# Autodesk Inventor assembly: POM_T5_03
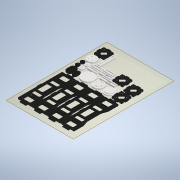
[picture p0: Inventor's stored thumbnail of the model, 180x180]
Saved by Autodesk Inventor 2020 (Build 240168000, 168)
## iProperties
Created: 2021-08-27
Part Number: POM_T5_03
Document SubType Name: Assembly
Designer: Masato
Author: Masato
## Documents named in this file (20)
- C:\Users\naoki\Documents\Inventor\CitBrains\git_clone\SUSTAINA_ver1_0\治具\SUSTAINA-OP\Cam\POM_T5_03.iam
- C:\Users\naoki\Documents\Inventor\CitBrains\git_clone\SUSTAINA_ver1_0\GFRP\SUSTAINA-OP\Cam\DisposableBoard.ipt
- C:\Users\naoki\Documents\Inventor\CitBrains\git_clone\SUSTAINA_ver1_0\GFRP\SUSTAINA-OP\UpperBody\Trunk\Trunk_chest_frame.ipt
- C:\Users\naoki\Documents\Inventor\CitBrains\git_clone\SUSTAINA_ver1_0\治具\SUSTAINA-OP\SandBlastingJig\Foot_front_frame_SandBlastingJig_back.ipt
- C:\Users\naoki\Documents\Inventor\CitBrains\git_clone\SUSTAINA_ver1_0\治具\SUSTAINA-OP\SandBlastingJig\Foot_front_frame_SandBlastingJig_front.ipt
- C:\Users\naoki\Documents\Inventor\CitBrains\git_clone\SUSTAINA_ver1_0\治具\SUSTAINA-OP\SandBlastingJig\Leg_joint_slider_frame_SandBlastingJig_axis_back.ipt
- C:\Users\naoki\Documents\Inventor\CitBrains\git_clone\SUSTAINA_ver1_0\治具\SUSTAINA-OP\SandBlastingJig\Leg_joint_slider_frame_SandBlastingJig_axis_front.ipt
- C:\Users\naoki\Documents\Inventor\CitBrains\git_clone\SUSTAINA_ver1_0\治具\SUSTAINA-OP\SandBlastingJig\Leg_joint_slider_frame_SandBlastingJig_slider_back.ipt
- C:\Users\naoki\Documents\Inventor\CitBrains\git_clone\SUSTAINA_ver1_0\治具\SUSTAINA-OP\SandBlastingJig\Leg_joint_slider_frame_SandBlastingJig_slider_front.ipt
- C:\Users\naoki\Documents\Inventor\CitBrains\git_clone\SUSTAINA_ver1_0\治具\SUSTAINA-OP\SandBlastingJig\Leg_joint_yaw_frame_SandBlastingJig.ipt
- C:\Users\naoki\Documents\Inventor\CitBrains\git_clone\SUSTAINA_ver1_0\治具\SUSTAINA-OP\SandBlastingJig\Outer_support_stand_SandBlastingJig.ipt
- C:\Users\naoki\Documents\Inventor\CitBrains\git_clone\SUSTAINA_ver1_0\治具\SUSTAINA-OP\SandBlastingJig\Shoulder_horn_frame_SandBlastingJig.ipt
- C:\Users\naoki\Documents\Inventor\CitBrains\git_clone\SUSTAINA_ver1_0\治具\SUSTAINA-OP\SandBlastingJig\Trunk_neck_frame_AND_Trunk_shoulder_frame_SandBlastingJig.ipt
- C:\Users\naoki\Documents\Inventor\CitBrains\git_clone\SUSTAINA_ver1_0\治具\SUSTAINA-OP\Jig\BackLink_diagonal_Jig.ipt
- C:\Users\naoki\Documents\Inventor\CitBrains\git_clone\SUSTAINA_ver1_0\治具\SUSTAINA-OP\Jig\Foot_root_block_Jig.ipt
- C:\Users\naoki\Documents\Inventor\CitBrains\git_clone\SUSTAINA_ver1_0\治具\SUSTAINA-OP\Jig\Leg_joint_yaw_frame_Jig.ipt
- C:\Users\naoki\Documents\Inventor\CitBrains\git_clone\SUSTAINA_ver1_0\治具\SUSTAINA-OP\Jig\Shoulder_horn_frame_Jig.ipt
- C:\Users\naoki\Documents\Inventor\CitBrains\git_clone\SUSTAINA_ver1_0\治具\SUSTAINA-OP\Jig\Trunk_lower_side_frame_Jig.ipt
- C:\Users\naoki\Documents\Inventor\CitBrains\git_clone\SUSTAINA_ver1_0\治具\SUSTAINA-OP\UpperBody\Arm\UpperArm_diagonal.ipt
- C:\Users\naoki\Documents\Inventor\CitBrains\git_clone\SUSTAINA_ver1_0\治具\SUSTAINA-OP\Jig\FrontLink_diagonal_Jig.ipt
## Components (25 placed, 19 different names)
1. DisposableBoard:1 — メイト:2, メイト:1, フラッシュ:1, フラッシュ:2, メイト:4, フラッシュ:3, フラッシュ:4, メイト:5, メイト:6, メイト:7, メイト:8, メイト:9, メイト:10, メイト:11, メイト:12, メイト:13, メイト:14, フラッシュ:5, 正接:9, 正接:10, 角度:1, 角度:2, メイト:16, メイト:17, メイト:18, メイト:20, メイト:21, 角度:3, メイト:31, フラッシュ:9, 正接:24, メイト:36, メイト:37, メイト:38, メイト:43
2. Foot_front_frame_SandBlastingJig_back:1 — メイト:14, 正接:11, 正接:13, 正接:14
3. Foot_front_frame_SandBlastingJig_front:1 — メイト:13, 正接:14, 正接:15, 正接:20, 正接:25
4. Leg_joint_slider_frame_SandBlastingJig_axis_back:1 — メイト:12, 正接:9, 正接:11, 正接:12, 正接:18
5. Leg_joint_slider_frame_SandBlastingJig_axis_front:1 — メイト:11, 正接:10, 正接:15, 正接:18
6. Leg_joint_slider_frame_SandBlastingJig_slider_back:1 — メイト:10, メイト:15, 正接:1, 正接:17
7. Leg_joint_slider_frame_SandBlastingJig_slider_front:1 — メイト:9, フラッシュ:5, メイト:15, 正接:12, 正接:13, 正接:16
8. Leg_joint_yaw_frame_SandBlastingJig:1 — メイト:8, 角度:2, 正接:24, 正接:25, 正接:27
9. Outer_support_stand_SandBlastingJig:1 — メイト:6, 正接:1, 正接:2, 正接:4, 正接:19
10. Shoulder_horn_frame_SandBlastingJig:1 — メイト:7, 正接:3, 正接:4, 正接:5, 角度:1, 正接:21, 正接:23
11. Trunk_neck_frame_AND_Trunk_shoulder_frame_SandBlastingJig:1 — メイト:5, 正接:5, 正接:6, 正接:22, 正接:26
12. BackLink_diagonal_Jig:1 — メイト:16, メイト:33, フラッシュ:12
13. Foot_root_block_Jig:1 — メイト:17, 正接:19, 正接:20, 角度:3, メイト:28, メイト:32, フラッシュ:10
14. Leg_joint_yaw_frame_Jig:1 — メイト:18, メイト:32, フラッシュ:10, メイト:44
15. Shoulder_horn_frame_Jig:1 — メイト:20, メイト:27, メイト:28, メイト:33, フラッシュ:12, メイト:42
16. Trunk_lower_side_frame_Jig:1 — メイト:21, 正接:21, 正接:22, 正接:23, メイト:27, メイト:40
17. UpperArm_diagonal:1 — メイト:31, フラッシュ:9, 正接:27, メイト:45
18. UpperArm_diagonal:2 — メイト:36, メイト:40, メイト:42
19. UpperArm_diagonal:3 — メイト:37, フラッシュ:11, メイト:41
20. UpperArm_diagonal:4 — メイト:38, メイト:39, 正接:26, フラッシュ:11, メイト:41
21. FrontLink_diagonal_Jig:1 — メイト:43, メイト:44, メイト:45
22. Trunk_chest_frame:1 — メイト:4, フラッシュ:3, フラッシュ:4, 正接:16, 正接:17
23. Trunk_chest_frame:3 — 正接:2
24. Trunk_chest_frame:4 — 正接:3, 正接:6
25. Trunk_chest_frame:5 — メイト:39
## Component patterns: (4 elements, first: Trunk_chest_frame:1)
## Relationships (71: Mate 34, Tangent 25, Flush 9, Angle 3)
- メイト:2 [Mate]: DisposableBoard:1
- メイト:1 [Mate]: DisposableBoard:1
- フラッシュ:1 [Flush]: DisposableBoard:1
- フラッシュ:2 [Flush]: DisposableBoard:1
- メイト:4 [Mate]: DisposableBoard:1 ↔ Trunk_chest_frame:1
- フラッシュ:3 [Flush] (2 mm): DisposableBoard:1 ↔ Trunk_chest_frame:1
- フラッシュ:4 [Flush] (2 mm): DisposableBoard:1 ↔ Trunk_chest_frame:1
- メイト:5 [Mate]: DisposableBoard:1 ↔ Trunk_neck_frame_AND_Trunk_shoulder_frame_SandBlastingJig:1
- メイト:6 [Mate]: DisposableBoard:1 ↔ Outer_support_stand_SandBlastingJig:1
- メイト:7 [Mate]: DisposableBoard:1 ↔ Shoulder_horn_frame_SandBlastingJig:1
- メイト:8 [Mate]: DisposableBoard:1 ↔ Leg_joint_yaw_frame_SandBlastingJig:1
- メイト:9 [Mate]: DisposableBoard:1 ↔ Leg_joint_slider_frame_SandBlastingJig_slider_front:1
- メイト:10 [Mate]: DisposableBoard:1 ↔ Leg_joint_slider_frame_SandBlastingJig_slider_back:1
- メイト:11 [Mate]: DisposableBoard:1 ↔ Leg_joint_slider_frame_SandBlastingJig_axis_front:1
- メイト:12 [Mate]: DisposableBoard:1 ↔ Leg_joint_slider_frame_SandBlastingJig_axis_back:1
- メイト:13 [Mate]: DisposableBoard:1 ↔ Foot_front_frame_SandBlastingJig_front:1
- メイト:14 [Mate]: DisposableBoard:1 ↔ Foot_front_frame_SandBlastingJig_back:1
- フラッシュ:5 [Flush] (2 mm): DisposableBoard:1 ↔ Leg_joint_slider_frame_SandBlastingJig_slider_front:1
- メイト:15 [Mate] (2.5 mm): Leg_joint_slider_frame_SandBlastingJig_slider_back:1 ↔ Leg_joint_slider_frame_SandBlastingJig_slider_front:1
- 正接:1 [Tangent] (2.5 mm): Leg_joint_slider_frame_SandBlastingJig_slider_back:1 ↔ Outer_support_stand_SandBlastingJig:1
- 正接:2 [Tangent] (2.5 mm): Outer_support_stand_SandBlastingJig:1 ↔ Trunk_chest_frame:3
- 正接:3 [Tangent] (2.5 mm): Shoulder_horn_frame_SandBlastingJig:1 ↔ Trunk_chest_frame:4
- 正接:4 [Tangent] (2.5 mm): Outer_support_stand_SandBlastingJig:1 ↔ Shoulder_horn_frame_SandBlastingJig:1
- 正接:5 [Tangent] (2.5 mm): Shoulder_horn_frame_SandBlastingJig:1 ↔ Trunk_neck_frame_AND_Trunk_shoulder_frame_SandBlastingJig:1
- 正接:6 [Tangent] (2.5 mm): Trunk_neck_frame_AND_Trunk_shoulder_frame_SandBlastingJig:1 ↔ Trunk_chest_frame:4
- 正接:9 [Tangent] (2 mm): DisposableBoard:1 ↔ Leg_joint_slider_frame_SandBlastingJig_axis_back:1
- 正接:10 [Tangent] (2 mm): DisposableBoard:1 ↔ Leg_joint_slider_frame_SandBlastingJig_axis_front:1
- 正接:11 [Tangent] (2.5 mm): Foot_front_frame_SandBlastingJig_back:1 ↔ Leg_joint_slider_frame_SandBlastingJig_axis_back:1
- 正接:12 [Tangent] (2.5 mm): Leg_joint_slider_frame_SandBlastingJig_axis_back:1 ↔ Leg_joint_slider_frame_SandBlastingJig_slider_front:1
- 正接:13 [Tangent] (2.5 mm): Foot_front_frame_SandBlastingJig_back:1 ↔ Leg_joint_slider_frame_SandBlastingJig_slider_front:1
- 正接:14 [Tangent] (2.5 mm): Foot_front_frame_SandBlastingJig_back:1 ↔ Foot_front_frame_SandBlastingJig_front:1
- 正接:15 [Tangent] (2.5 mm): Foot_front_frame_SandBlastingJig_front:1 ↔ Leg_joint_slider_frame_SandBlastingJig_axis_front:1
- 正接:16 [Tangent] (2.5 mm): Leg_joint_slider_frame_SandBlastingJig_slider_front:1 ↔ Trunk_chest_frame:1
- 正接:17 [Tangent] (2.5 mm): Leg_joint_slider_frame_SandBlastingJig_slider_back:1 ↔ Trunk_chest_frame:1
- 正接:18 [Tangent] (2.5 mm): Leg_joint_slider_frame_SandBlastingJig_axis_back:1 ↔ Leg_joint_slider_frame_SandBlastingJig_axis_front:1
- 角度:1 [Angle] (0 deg): DisposableBoard:1 ↔ Shoulder_horn_frame_SandBlastingJig:1
- 角度:2 [Angle] (0 deg): DisposableBoard:1 ↔ Leg_joint_yaw_frame_SandBlastingJig:1
- メイト:16 [Mate]: DisposableBoard:1 ↔ BackLink_diagonal_Jig:1
- メイト:17 [Mate]: DisposableBoard:1 ↔ Foot_root_block_Jig:1
- メイト:18 [Mate]: DisposableBoard:1 ↔ Leg_joint_yaw_frame_Jig:1
- メイト:20 [Mate]: DisposableBoard:1 ↔ Shoulder_horn_frame_Jig:1
- メイト:21 [Mate]: DisposableBoard:1 ↔ Trunk_lower_side_frame_Jig:1
- 正接:19 [Tangent] (2.5 mm): Outer_support_stand_SandBlastingJig:1 ↔ Foot_root_block_Jig:1
- 正接:20 [Tangent] (2.5 mm): Foot_front_frame_SandBlastingJig_front:1 ↔ Foot_root_block_Jig:1
- 角度:3 [Angle] (180 deg): DisposableBoard:1 ↔ Foot_root_block_Jig:1
- 正接:21 [Tangent] (2.5 mm): Shoulder_horn_frame_SandBlastingJig:1 ↔ Trunk_lower_side_frame_Jig:1
- 正接:22 [Tangent] (2.5 mm): Trunk_neck_frame_AND_Trunk_shoulder_frame_SandBlastingJig:1 ↔ Trunk_lower_side_frame_Jig:1
- 正接:23 [Tangent]: Shoulder_horn_frame_SandBlastingJig:1 ↔ Trunk_lower_side_frame_Jig:1
- メイト:27 [Mate] (2.5 mm): Shoulder_horn_frame_Jig:1 ↔ Trunk_lower_side_frame_Jig:1
- メイト:28 [Mate] (2.5 mm): Foot_root_block_Jig:1 ↔ Shoulder_horn_frame_Jig:1
- メイト:31 [Mate]: DisposableBoard:1 ↔ UpperArm_diagonal:1
- フラッシュ:9 [Flush] (2 mm): DisposableBoard:1 ↔ UpperArm_diagonal:1
- 正接:24 [Tangent] (2 mm): DisposableBoard:1 ↔ Leg_joint_yaw_frame_SandBlastingJig:1
- 正接:25 [Tangent] (2.5 mm): Foot_front_frame_SandBlastingJig_front:1 ↔ Leg_joint_yaw_frame_SandBlastingJig:1
- メイト:32 [Mate] (2.5 mm): Foot_root_block_Jig:1 ↔ Leg_joint_yaw_frame_Jig:1
- フラッシュ:10 [Flush]: Foot_root_block_Jig:1 ↔ Leg_joint_yaw_frame_Jig:1
- メイト:33 [Mate] (2.5 mm): BackLink_diagonal_Jig:1 ↔ Shoulder_horn_frame_Jig:1
- メイト:36 [Mate]: DisposableBoard:1 ↔ UpperArm_diagonal:2
- メイト:37 [Mate]: DisposableBoard:1 ↔ UpperArm_diagonal:3
- メイト:38 [Mate]: DisposableBoard:1 ↔ UpperArm_diagonal:4
- メイト:39 [Mate] (2.5 mm): UpperArm_diagonal:4 ↔ Trunk_chest_frame:5
- 正接:26 [Tangent] (2.5 mm): Trunk_neck_frame_AND_Trunk_shoulder_frame_SandBlastingJig:1 ↔ UpperArm_diagonal:4
- フラッシュ:11 [Flush]: UpperArm_diagonal:3 ↔ UpperArm_diagonal:4
- メイト:40 [Mate] (2.5 mm): Trunk_lower_side_frame_Jig:1 ↔ UpperArm_diagonal:2
- フラッシュ:12 [Flush]: BackLink_diagonal_Jig:1 ↔ Shoulder_horn_frame_Jig:1
- 正接:27 [Tangent] (2.5 mm): Leg_joint_yaw_frame_SandBlastingJig:1 ↔ UpperArm_diagonal:1
- メイト:41 [Mate] (2.5 mm): UpperArm_diagonal:3 ↔ UpperArm_diagonal:4
- メイト:42 [Mate] (2.5 mm): Shoulder_horn_frame_Jig:1 ↔ UpperArm_diagonal:2
- メイト:43 [Mate]: DisposableBoard:1 ↔ FrontLink_diagonal_Jig:1
- メイト:44 [Mate] (2.5 mm): Leg_joint_yaw_frame_Jig:1 ↔ FrontLink_diagonal_Jig:1
- メイト:45 [Mate] (2.5 mm): UpperArm_diagonal:1 ↔ FrontLink_diagonal_Jig:1
